# Autodesk Inventor assembly: Center of Gravity Shifter Assembly
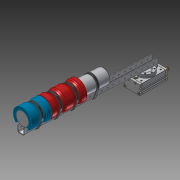
[picture p0: Inventor's stored thumbnail of the model, 180x180]
Saved by Autodesk Inventor 2014 SP1 (Build 180222100, 222)
## iProperties
Created: 2013-12-16
Part Number: Center of Gravity Shifter Assembly
Document SubType Name: Assembly
Designer: Moses
Mass: 3972.82 g
Surface Area: 3949.62 cm^2
Volume: 2210.35 cm^3
Density: 1.79737 g/cm^3
Author: Moses
## Documents named in this file (11)
- C:\Users\Moses\Documents\Inventor\Sally Rebuild\Rebuild Sally\Center of Gravity Shifter Assembly.iam
- C:\Users\Moses\Documents\Inventor\Sally Rebuild\Rebuild Sally\Center of Mass Shifter Arm - Chassis_Channel_AndyMark.ipt
- C:\Users\Moses\Documents\Inventor\Sally Rebuild\Rebuild Sally\0.25x20 Washer.ipt
- C:\Users\Moses\Documents\Inventor\Sally Rebuild\Rebuild Sally\Standard High-Strength Steel Cap Screw 0.25-20 Thread\Fully Threaded\0.750 in 92620A540\92620A540.ipt
- C:\Users\Moses\Documents\Inventor\Sally Rebuild\Rebuild Sally\Standard High-Strength Steel Cap Screw 0.25-20 Thread\Thread Length 0.75 - 1 in\2.500 in 91257A552\91257A552.ipt
- C:\Users\Moses\Documents\Inventor\Sally Rebuild\Rebuild Sally\Climber Extra Weight Cylinder.ipt
- C:\Users\Moses\Documents\Inventor\Sally Rebuild\Rebuild Sally\SMC MSQ Rotary Pneumatic Rack and Pinion Rotary Table Block.iam
- C:\Users\Moses\Documents\Inventor\Sally Rebuild\Rebuild Sally\Foam Weight Shifter Pad 2.ipt
- C:\Users\Moses\Documents\Inventor\Sally Rebuild\Rebuild Sally\Foam Weight Shifter Pad 1.ipt
- C:\Users\Moses\Documents\Inventor\Sally Rebuild\Rebuild Sally\Weight Shifter Tension Strap.ipt
- C:\Users\Moses\Documents\Inventor\Sally Rebuild\Rebuild Sally\Weight Shifter Tension Strap 2.ipt
## Components (26 placed, 10 different names)
1. SMC MSQ Rotary Pneumatic Rack and Pinion Rotary Table Block:1 [sub-assembly] — Mate:1, Mate:2, Angle:1, Mate:3, Insert:13, Insert:14
2. Center of Mass Shifter Arm - Chassis_Channel_AndyMark:1 — Mate:1, Mate:2, Angle:1, Mate:3, Insert:1, Insert:10, Tangent:1, Tangent:2, Tangent:3, Tangent:4, Flush:1, Angle:2, Mate:11, Mate:17, Mate:18, Mate:19
3. 0.25x20 Washer:1 — Insert:1, Insert:2
4. 0.25x20 Washer:2 — Insert:2, Insert:3
5. 0.25x20 Washer:3 — Insert:3, Insert:4
6. 0.25x20 Washer:4 — Insert:4, Insert:5
7. 0.25x20 Washer:5 — Insert:5, Insert:11
8. 0.25x20 Washer:6 — Insert:10
9. 0.25x20 Washer:7
10. 0.25x20 Washer:8
11. 0.25x20 Washer:9
12. 0.25x20 Washer:10 — Insert:12
13. 92620A540:1 — Insert:11
14. 92620A540:2 — Insert:12
15. 0.25x20 Washer:11 — Insert:13, Insert:15
16. 0.25x20 Washer:12 — Insert:14, Insert:16
17. 91257A552:1 — Insert:15
18. 91257A552:2 — Insert:16
19. Climber Extra Weight Cylinder:1 — Tangent:3, Tangent:4, Flush:1, Mate:4, Mate:5, Mate:6, Flush:2
20. Climber Extra Weight Cylinder:2 — Tangent:1, Tangent:2, Mate:4, Mate:5, Mate:7, Mate:20, Flush:5
21. Foam Weight Shifter Pad 1:1 — Mate:6, Flush:2, Flush:4, Angle:2, Mate:8, Mate:9, Mate:10, Mate:12
22. Foam Weight Shifter Pad 2:1 — Mate:7, Mate:8, Flush:4, Mate:13, Mate:14, Mate:15, Mate:16
23. Weight Shifter Tension Strap:1 — Mate:9, Mate:10, Mate:11, Mate:12
24. Weight Shifter Tension Strap:2 — Mate:13, Mate:14, Mate:17
25. Weight Shifter Tension Strap:3 — Mate:15, Mate:16, Mate:18
26. Weight Shifter Tension Strap 2:1 — Mate:19, Mate:20, Flush:5
## Relationships (46: Mate 20, Insert 16, Tangent 4, Flush 4, Angle 2)
- Mate:1: SMC MSQ Rotary Pneumatic Rack and Pinion Rotary Table Block:1 ↔ Center of Mass Shifter Arm - Chassis_Channel_AndyMark:1
- Mate:2: SMC MSQ Rotary Pneumatic Rack and Pinion Rotary Table Block:1 ↔ Center of Mass Shifter Arm - Chassis_Channel_AndyMark:1
- Angle:1 (-2.5 deg): SMC MSQ Rotary Pneumatic Rack and Pinion Rotary Table Block:1 ↔ Center of Mass Shifter Arm - Chassis_Channel_AndyMark:1
- Mate:3: SMC MSQ Rotary Pneumatic Rack and Pinion Rotary Table Block:1 ↔ Center of Mass Shifter Arm - Chassis_Channel_AndyMark:1
- Insert:1: Center of Mass Shifter Arm - Chassis_Channel_AndyMark:1 ↔ 0.25x20 Washer:1
- Insert:2: 0.25x20 Washer:1 ↔ 0.25x20 Washer:2
- Insert:3: 0.25x20 Washer:2 ↔ 0.25x20 Washer:3
- Insert:4: 0.25x20 Washer:3 ↔ 0.25x20 Washer:4
- Insert:5: 0.25x20 Washer:4 ↔ 0.25x20 Washer:5
- [Insert]: 0.25x20 Washer:6 ↔ 0.25x20 Washer:7
- [Insert]: 0.25x20 Washer:7 ↔ 0.25x20 Washer:8
- [Insert]: 0.25x20 Washer:8 ↔ 0.25x20 Washer:9
- [Insert]: 0.25x20 Washer:9 ↔ 0.25x20 Washer:10
- Insert:10: Center of Mass Shifter Arm - Chassis_Channel_AndyMark:1 ↔ 0.25x20 Washer:6
- Insert:11: 0.25x20 Washer:5 ↔ 92620A540:1
- Insert:12: 0.25x20 Washer:10 ↔ 92620A540:2
- Insert:13: SMC MSQ Rotary Pneumatic Rack and Pinion Rotary Table Block:1 ↔ 0.25x20 Washer:11
- Insert:14: SMC MSQ Rotary Pneumatic Rack and Pinion Rotary Table Block:1 ↔ 0.25x20 Washer:12
- Insert:15: 0.25x20 Washer:11 ↔ 91257A552:1
- Insert:16: 0.25x20 Washer:12 ↔ 91257A552:2
- Tangent:1: Center of Mass Shifter Arm - Chassis_Channel_AndyMark:1 ↔ Climber Extra Weight Cylinder:2
- Tangent:2: Center of Mass Shifter Arm - Chassis_Channel_AndyMark:1 ↔ Climber Extra Weight Cylinder:2
- Tangent:3: Center of Mass Shifter Arm - Chassis_Channel_AndyMark:1 ↔ Climber Extra Weight Cylinder:1
- Tangent:4: Center of Mass Shifter Arm - Chassis_Channel_AndyMark:1 ↔ Climber Extra Weight Cylinder:1
- Flush:1 (6.35 mm): Center of Mass Shifter Arm - Chassis_Channel_AndyMark:1 ↔ Climber Extra Weight Cylinder:1
- Mate:4 (3.175 mm): Climber Extra Weight Cylinder:1 ↔ Climber Extra Weight Cylinder:2
- Mate:5: Climber Extra Weight Cylinder:1 ↔ Climber Extra Weight Cylinder:2
- Mate:6: Climber Extra Weight Cylinder:1 ↔ Foam Weight Shifter Pad 1:1
- Mate:7: Climber Extra Weight Cylinder:2 ↔ Foam Weight Shifter Pad 2:1
- Flush:2: Climber Extra Weight Cylinder:1 ↔ Foam Weight Shifter Pad 1:1
- Mate:8 (3.175 mm): Foam Weight Shifter Pad 1:1 ↔ Foam Weight Shifter Pad 2:1
- Flush:4: Foam Weight Shifter Pad 1:1 ↔ Foam Weight Shifter Pad 2:1
- Angle:2 (135 deg): Center of Mass Shifter Arm - Chassis_Channel_AndyMark:1 ↔ Foam Weight Shifter Pad 1:1
- Mate:9: Foam Weight Shifter Pad 1:1 ↔ Weight Shifter Tension Strap:1
- Mate:10: Foam Weight Shifter Pad 1:1 ↔ Weight Shifter Tension Strap:1
- Mate:11: Center of Mass Shifter Arm - Chassis_Channel_AndyMark:1 ↔ Weight Shifter Tension Strap:1
- Mate:12: Foam Weight Shifter Pad 1:1 ↔ Weight Shifter Tension Strap:1
- Mate:13: Foam Weight Shifter Pad 2:1 ↔ Weight Shifter Tension Strap:2
- Mate:14: Foam Weight Shifter Pad 2:1 ↔ Weight Shifter Tension Strap:2
- Mate:15: Foam Weight Shifter Pad 2:1 ↔ Weight Shifter Tension Strap:3
- Mate:16: Foam Weight Shifter Pad 2:1 ↔ Weight Shifter Tension Strap:3
- Mate:17: Center of Mass Shifter Arm - Chassis_Channel_AndyMark:1 ↔ Weight Shifter Tension Strap:2
- Mate:18: Center of Mass Shifter Arm - Chassis_Channel_AndyMark:1 ↔ Weight Shifter Tension Strap:3
- Mate:19: Center of Mass Shifter Arm - Chassis_Channel_AndyMark:1 ↔ Weight Shifter Tension Strap 2:1
- Mate:20: Climber Extra Weight Cylinder:2 ↔ Weight Shifter Tension Strap 2:1
- Flush:5 (50.8 mm): Climber Extra Weight Cylinder:2 ↔ Weight Shifter Tension Strap 2:1
## Named parameters: d9_d5 = 0 mm, d10_d6 = 0 mm, d11_d7 = 0 mm, d12_d8 = 0 mm
